# Autodesk Inventor assembly: wheelAssembly
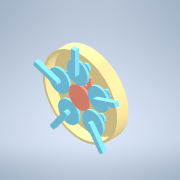
[picture p0: Inventor's stored thumbnail of the model, 180x180]
Saved by Autodesk Inventor 2020.1 (Build 241239000, 239)
## iProperties
Created: 2020-01-18
Part Number: wheelAssembly
Document SubType Name: Assembly
Designer: Ali
Author: Ali
## Documents named in this file (7)
- F:\Inventor_Projects\ARCS\ASSEMBLIES\wheelAssembly.iam
- F:\Inventor_Projects\ARCS\PARTS\wheel.ipt
- F:\Inventor_Projects\ARCS\PARTS\innerGear.ipt
- F:\Inventor_Projects\ARCS\PARTS\outerGear.ipt
- F:\Inventor_Projects\ARCS\PARTS\bearing.ipt
- F:\Inventor_Projects\ARCS\PARTS\block.ipt
- F:\Inventor_Projects\ARCS\Excel\New_Parameters.xlsx
## Components (9 placed, 5 different names)
1. wheel:1 — Insert:1, Insert:2, Insert:3, Mate:1, Mate:2
2. innerGear:1 — Insert:1
3. bearing:1 — Insert:3
4. block:1 — Mate:1, Mate:2
5. outerGear:1 — Insert:2
6. outerGear:2
7. outerGear:3
8. outerGear:4
9. outerGear:5
## Component patterns: (5 elements, first: outerGear:1)
## Relationships (5: Insert 3, Mate 2)
- Insert:1 (-5 mm): wheel:1 ↔ innerGear:1
- Insert:2: wheel:1 ↔ outerGear:1
- Insert:3: wheel:1 ↔ bearing:1
- Mate:1: wheel:1 ↔ block:1
- Mate:2: wheel:1 ↔ block:1
## Named parameters: Wheel_Related_W_ = 0, W_innerDiameter = 35 mm, W_innerDepth = 4.5 mm, W_wallThickness = 1 mm, W_holesClearance = 0.3 mm, W_outerGearHoleDiameter = 2.1 mm, W_innerGearHoleDiameter = 5.1 mm, TempSpotReserved7 = 0 mm, TempSpotReserved8 = 0 mm, TempSpotReserved9 = 0 mm, TempSpotReserved10 = 0 mm, TempSpotReserved11 = 0 mm, TempSpotReserved12 = 0 mm, TempSpotReserved13 = 0 mm, TempSpotReserved14 = 0 mm, TempSpotReserved15 = 0 mm, TempSpotReserved16 = 0 mm, TempSpotReserved17 = 0 mm, TempSpotReserved18 = 0 mm, TempSpotReserved19 = 0 mm, TempSpotReserved20 = 0 mm, Inner_Gear_Related_IG_ = 0, IG_shaftDiameter = 2.5 mm, IG_gearDiameter = 10 mm, IG_shaftLength = 10 mm, IG_gearThickness = 1 mm, TempSpotReserved25 = 0 mm, TempSpotReserved26 = 0 mm, TempSpotReserved27 = 0 mm, TempSpotReserved28 = 0 mm, TempSpotReserved29 = 0 mm, TempSpotReserved30 = 0 mm, TempSpotReserved31 = 0 mm, TempSpotReserved32 = 0 mm, TempSpotReserved33 = 0 mm, TempSpotReserved34 = 0 mm, TempSpotReserved35 = 0 mm, TempSpotReserved36 = 0 mm, TempSpotReserved37 = 0 mm, TempSpotReserved38 = 0 mm, TempSpotReserved39 = 0 mm, TempSpotReserved40 = 0 mm, Outer_Gear_Related_OG_ = 0, OG_distanceFromCenter = 10 mm, OG_shaftDiameter = 1.5 mm, OG_gearDiameter = 10 mm, OG_numberOfGears = 5, OG_shaftLength = 5 mm, OG_gearThickness = 1 mm, TempSpotReserved47 = 0 mm, TempSpotReserved48 = 0 mm, TempSpotReserved49 = 0 mm, TempSpotReserved50 = 0 mm, TempSpotReserved51 = 0 mm, TempSpotReserved52 = 0 mm, TempSpotReserved53 = 0 mm, TempSpotReserved54 = 0 mm, TempSpotReserved55 = 0 mm, TempSpotReserved56 = 0 mm, TempSpotReserved57 = 0 mm, TempSpotReserved58 = 0 mm, TempSpotReserved59 = 0 mm, TempSpotReserved60 = 0 mm, Leg_Extensions_Related_LE_ = 0, LE_baseDiameter = 2 mm, LE_maxLength = 10.64459 mm, LE_thickness = 2 mm, IG_ratioToOuterGear = 1, B_bearingThickness = 1 mm, TempSpotReserved43 = 0 mm, TempSpotReserved45 = 0 mm, Thisisatest = 25.4 mm, TempSpotReserved46 = 0 mm, TempSpotReserved44 = 0 mm, LE_offsetAboveOuterGear = 0 mm, Bearing_Related_B_ = 0, TempSpotReserved42 = 0 mm, OG_skirtOffset = 1 mm, OG_skirtThickness = 1 mm, IG_skirtThickness = 0.5 mm, IG_skirtOffset = 1.5 mm, IG_extentionLength = 7 mm, IG_extentionThickness = 1 mm, IG_slitWidth = 1.5 mm, IG_slitlength = 4 mm
